# Autodesk Inventor assembly: 1x1_asm_main
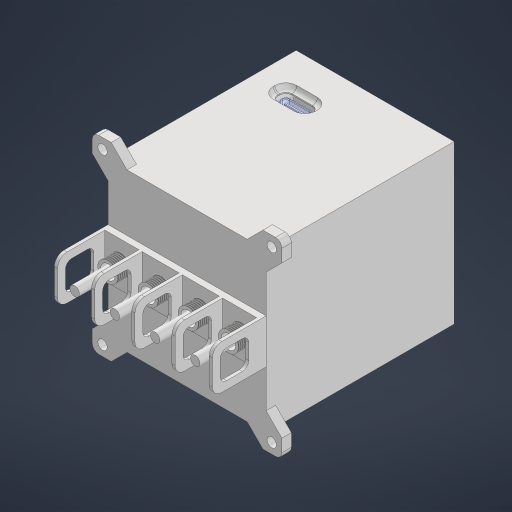
[picture p0: Inventor's stored thumbnail of the model, 512x512]
Saved by Autodesk Inventor 2024 (Build 280153000, 153)
## iProperties
Created: 2026-04-07
Part Number: 1x1_asm_main
Document SubType Name: Assembly
Designer: schar
Author: schar
## Documents named in this file (6)
- C:\Users\schar\Desktop\MHIPS\models\tiles\1x1\lvl301x01_4t\1x1_asm_main.iam
- C:\Users\schar\Desktop\MHIPS\models\BusPlate\BusPlate.ipt
- C:\Users\schar\Desktop\MHIPS\models\tiles\1x1\lvl301x01_4t\casing_1x1_lvl3.ipt
- C:\Users\schar\Desktop\MHIPS\models\tiles\1x1\lvl301x01_4t\backplate.ipt
- C:\Users\schar\Desktop\MHIPS\models\switches\APEM_5236CDB.ipt
- C:\Users\schar\Desktop\MHIPS\models\tiles\1x1\lvl301x01_4t\protector_small1x1.ipt
## Components (8 placed, 5 different names)
1. casing_1x1_lvl3:1 — Mate:4, Flush:1, Mate:5, Angle:1, Angle:2, Angle:3, Angle:4, Mate:6, Mate:7, Mate:8, Mate:9, Mate:10, Mate:11, Mate:12, Mate:13, Flush:2, Mate:14, Mate:15, Mate:16
2. APEM_5236CDB:1 — Angle:1, Mate:6, Mate:7
3. APEM_5236CDB:2 — Angle:2, Mate:8, Mate:9
4. APEM_5236CDB:3 — Angle:3, Mate:10, Mate:11
5. APEM_5236CDB:4 — Angle:4, Mate:12, Mate:13
6. protector_small1x1:1 — Flush:2
7. BusPlate:1 — Mate:14, Mate:15, Mate:16, Mate:17, Mate:18, Mate:19
8. backplate:1 — Mate:17, Mate:18, Mate:19
## Relationships (22: Mate 16, Angle 4, Flush 2)
- Mate:4: casing_1x1_lvl3:1
- Flush:1: casing_1x1_lvl3:1
- Mate:5: casing_1x1_lvl3:1
- Angle:1 (0 deg): casing_1x1_lvl3:1 ↔ APEM_5236CDB:1
- Angle:2 (0 deg): casing_1x1_lvl3:1 ↔ APEM_5236CDB:2
- Angle:3 (0 deg): casing_1x1_lvl3:1 ↔ APEM_5236CDB:3
- Angle:4 (0 deg): casing_1x1_lvl3:1 ↔ APEM_5236CDB:4
- Mate:6: casing_1x1_lvl3:1 ↔ APEM_5236CDB:1
- Mate:7: casing_1x1_lvl3:1 ↔ APEM_5236CDB:1
- Mate:8: casing_1x1_lvl3:1 ↔ APEM_5236CDB:2
- Mate:9: casing_1x1_lvl3:1 ↔ APEM_5236CDB:2
- Mate:10: casing_1x1_lvl3:1 ↔ APEM_5236CDB:3
- Mate:11: casing_1x1_lvl3:1 ↔ APEM_5236CDB:3
- Mate:12: casing_1x1_lvl3:1 ↔ APEM_5236CDB:4
- Mate:13: casing_1x1_lvl3:1 ↔ APEM_5236CDB:4
- Flush:2: casing_1x1_lvl3:1 ↔ protector_small1x1:1
- Mate:14 (0.2 mm): casing_1x1_lvl3:1 ↔ BusPlate:1
- Mate:15: casing_1x1_lvl3:1 ↔ BusPlate:1
- Mate:16 (3.16 mm): casing_1x1_lvl3:1 ↔ BusPlate:1
- Mate:17: BusPlate:1 ↔ backplate:1
- Mate:18: BusPlate:1 ↔ backplate:1
- Mate:19: BusPlate:1 ↔ backplate:1
